# Autodesk Inventor assembly: hintererAufbau
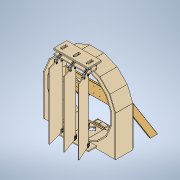
[picture p0: Inventor's stored thumbnail of the model, 180x180]
Saved by Autodesk Inventor 2020.3 (Build 243373000, 373)
## iProperties
Created: 2021-02-11
Part Number: hintererAufbau
Document SubType Name: Assembly
Designer: Stefan
Author: Stefan
## Documents named in this file (31)
- D:\Stefan\Schule\HTL\Diplomarbeit\git\Inventor\hintererAufbau\hintererAufbau.iam
- D:\Stefan\Schule\HTL\Diplomarbeit\git\Inventor\hintererAufbau\Hauptplatte.ipt
- D:\Stefan\Schule\HTL\Diplomarbeit\git\Inventor\hintererAufbau\InnenUnten.ipt
- D:\Stefan\Schule\HTL\Diplomarbeit\git\Inventor\hintererAufbau\aussenOben.ipt
- D:\Stefan\Schule\HTL\Diplomarbeit\git\Inventor\hintererAufbau\PlatteInnenEineSeite.ipt
- D:\Stefan\Schule\HTL\Diplomarbeit\git\Inventor\hintererAufbau\PlatteInnenzweiSeiten.ipt
- D:\Stefan\Schule\HTL\Diplomarbeit\git\Inventor\hintererAufbau\PlatteAussenEineSeite.ipt
- D:\Stefan\Schule\HTL\Diplomarbeit\git\Inventor\hintererAufbau\PlatteAussenZweiSeiten.ipt
- D:\Stefan\Schule\HTL\Diplomarbeit\git\Inventor\hintererAufbau\PlatteAußenGross.ipt
- D:\Stefan\Schule\HTL\Diplomarbeit\git\Inventor\3D-Druck\Fahnen_Halter_hauptteil.ipt
- D:\Stefan\Schule\HTL\Diplomarbeit\git\Inventor\3D-Druck\Fahnen_Halter_rechteck.ipt
- D:\Stefan\Schule\HTL\Diplomarbeit\git\Inventor\3D-Druck\Fahnen_Halter_obenTeileServo.ipt
- D:\Stefan\Schule\HTL\Diplomarbeit\git\Inventor\hintererAufbau\FahneHolz.ipt
- C:\Users\Stefan\Documents\Inventor\Content Center Files\R2020\de-DE\DIN EN 24 017\ISO 4017 - M5 x 30DIN EN.ipt
- C:\Users\Stefan\Documents\Inventor\Content Center Files\R2020\de-DE\ISO 4032(1)\ISO 4032 - M5DIN EN.ipt
- C:\Users\Stefan\Documents\Inventor\Content Center Files\R2020\de-DE\DIN EN 24 017\ISO 4017 - M5 x 40DIN EN.ipt
- D:\Stefan\Schule\HTL\Diplomarbeit\git\Inventor\hintererAufbau\VerstaerkungHintenMitte.ipt
- D:\Stefan\Schule\HTL\Diplomarbeit\git\Inventor\hintererAufbau\VerstaerkungHintenUnten.ipt
- D:\Stefan\Schule\HTL\Diplomarbeit\git\Inventor\hintererAufbau\VerstaerkungHintenSchraeg.ipt
- D:\Stefan\Schule\HTL\Diplomarbeit\git\Inventor\hintererAufbau\HalterungServoHochSeitlich2.ipt
- D:\Stefan\Schule\HTL\Diplomarbeit\git\Inventor\hintererAufbau\HalterungServosHochSeitlich.ipt
- D:\Stefan\Schule\HTL\Diplomarbeit\git\Inventor\hintererAufbau\HolzServoHalterHochLang.ipt
- D:\Stefan\Schule\HTL\Diplomarbeit\git\Inventor\hintererAufbau\HolzServoHalterMainPlatte1.ipt
- D:\Stefan\Schule\HTL\Diplomarbeit\git\Inventor\hintererAufbau\HolzServoHalterHinten.ipt
- D:\Stefan\Schule\HTL\Diplomarbeit\git\Inventor\Servo.ipt
- D:\Stefan\Schule\HTL\Diplomarbeit\git\Inventor\3D-Druck\Spacer_Relay v2.ipt
- D:\Stefan\Schule\HTL\Diplomarbeit\git\Inventor\hintererAufbau\VerstaerkungUnten.ipt
- D:\Stefan\Schule\HTL\Diplomarbeit\git\Inventor\hintererAufbau\KabelBoxPlatteLang.ipt
- D:\Stefan\Schule\HTL\Diplomarbeit\git\Inventor\hintererAufbau\KabelBoxPlatteKurz.ipt
- D:\Stefan\Schule\HTL\Diplomarbeit\git\Inventor\hintererAufbau\KabelBoxDeckel.ipt
- D:\Stefan\Schule\HTL\Diplomarbeit\git\Inventor\hintererAufbau\InventorOnlyInvisibleSchanierl.ipt
## Components (135 placed, 30 different names)
1. Hauptplatte:1 — Passend:1, Passend:3, Passend:5, Passend:6, Passend:9, Fluchtend:7, Passend:36, Passend:37, Fluchtend:14, Fluchtend:15, Fluchtend:16, Passend:46, Passend:47, Fluchtend:17, Passend:48, Passend:49, Passend:52, Passend:147, Fluchtend:66, Fluchtend:67
2. Hauptplatte:2 — Passend:2, Passend:4, Fluchtend:1, Passend:7, Fluchtend:2, Passend:8, Fluchtend:3, Passend:11, Passend:12, Passend:13, Passend:14, Passend:15, Passend:16, Passend:17, Passend:18, Fluchtend:4, Passend:19, Fluchtend:5, Passend:20, Passend:21, Fluchtend:6, Passend:22, Passend:23, Passend:24, Passend:25, Fluchtend:8, Passend:26, Passend:27, Fluchtend:9, Passend:28, Passend:29, Fluchtend:10, Passend:30, Passend:31, Passend:32, Fluchtend:11, Passend:33, Fluchtend:12, Passend:34, Passend:35, Fluchtend:13, Passend:38, Passend:39, Passend:40, Passend:41, Passend:42, Passend:43, Passend:44, Passend:45, Fluchtend:18, Passend:50, Passend:51, Fluchtend:19, Passend:99, Fluchtend:28, Fluchtend:29, Fluchtend:30, Passend:135, Fluchtend:52, Passend:148
3. InnenUnten:1 — Passend:1, Passend:2, Passend:3, Passend:4, Fluchtend:1, Passend:5, Passend:10, Passend:55, Passend:56, Passend:58, Passend:62, Passend:63, Passend:64, Passend:131, Passend:132, Passend:133, Passend:134
4. aussenOben:1 — Passend:6, Passend:7, Fluchtend:2, Passend:8, Passend:70, Passend:71, Passend:72, Passend:73, Passend:74, Passend:75, Passend:78, Passend:79, Passend:80, Passend:124, Fluchtend:49, Fluchtend:50
5. FahneHolz:1 — Passend:85, Passend:86, Passend:87, Passend:88
6. FahneHolz:2 — Passend:89, Passend:90, Passend:91, Passend:92
7. FahneHolz:3 — Passend:93, Passend:94, Passend:95, Passend:96
8. VerstaerkungHintenMitte:1 — Passend:97, Passend:98, Fluchtend:24, Fluchtend:25, Fluchtend:26, Fluchtend:27, Passend:99, Fluchtend:28, Passend:100, Fluchtend:31, Passend:101, Fluchtend:33
9. VerstaerkungHintenUnten:1 — Passend:98, Fluchtend:25, Fluchtend:27, Fluchtend:29, Fluchtend:34
10. VerstaerkungHintenUnten:2 — Passend:97, Fluchtend:24, Fluchtend:26, Fluchtend:30, Passend:136
11. VerstaerkungHintenSchraeg:1 — Passend:100, Fluchtend:31, Fluchtend:32
12. VerstaerkungHintenSchraeg:2 — Passend:101, Fluchtend:33, Fluchtend:34
13. HalterungServoHochSeitlich2:1 — Passend:104, Fluchtend:39, Passend:105, Passend:106, Passend:109, Fluchtend:42, Passend:111
14. HalterungServosHochSeitlich:1 — Passend:102, Fluchtend:35, Fluchtend:36, Fluchtend:50, Fluchtend:46
15. HolzServoHalterHochLang:1 — Passend:102, Fluchtend:35, Fluchtend:36, Passend:103, Fluchtend:37, Fluchtend:38, Passend:104, Fluchtend:39, Passend:105, Passend:106, Passend:107, Fluchtend:40, Passend:108, Passend:113, Fluchtend:49
16. HolzServoHalterMainPlatte1:1 — Fluchtend:47, Fluchtend:48, Passend:114, Passend:128, Passend:129, Passend:130
17. HalterungServoHochSeitlich2:2 — Passend:107, Fluchtend:40, Passend:108, Passend:110, Fluchtend:41, Fluchtend:43
18. HalterungServosHochSeitlich:2 — Passend:103, Fluchtend:37, Fluchtend:38
19. HolzServoHalterMainPlatte1:2 — Passend:112, Passend:113, Fluchtend:46, Fluchtend:47, Fluchtend:48, Passend:114, Passend:115, Passend:118, Passend:119, Fluchtend:51, Passend:125, Passend:126, Passend:127
20. HolzServoHalterHinten:1 — Passend:109, Passend:110, Fluchtend:41, Fluchtend:42, Passend:111, Fluchtend:43, Passend:112, Passend:124, Fluchtend:51
21. Servo:1 — Passend:115, Passend:125, Passend:128
22. Servo:2 — Passend:118, Passend:126, Passend:129
23. Servo:3 — Passend:119, Passend:127, Passend:130
24. Spacer_Relay v2:1 — Passend:131, Passend:134
25. Spacer_Relay v2:2 — Passend:132, Passend:133
26. VerstaerkungUnten:1 — Passend:135, Fluchtend:52, Passend:136, Passend:146, Fluchtend:63
27. KabelBoxPlatteLang:1 — Passend:138, Fluchtend:55, Fluchtend:56, Fluchtend:58, Passend:140, Passend:144
28. KabelBoxPlatteLang:2 — Passend:137, Fluchtend:53, Fluchtend:54, Passend:139, Fluchtend:57, Passend:146, Fluchtend:63
29. KabelBoxPlatteKurz:1 — Passend:139, Fluchtend:57, Fluchtend:58, Passend:142, Fluchtend:65
30. KabelBoxPlatteKurz:2 — Passend:137, Fluchtend:53, Fluchtend:54, Passend:138, Fluchtend:55, Fluchtend:56, Passend:145
31. KabelBoxDeckel:1 — Passend:140, Passend:141, Fluchtend:59, Fluchtend:60
32. InventorOnlyInvisibleSchanierl:1 — Passend:141, Fluchtend:59, Fluchtend:60, Passend:142
33. InventorOnlyInvisibleSchanierl:2 — Passend:143, Fluchtend:61, Fluchtend:62, Passend:145
34. KabelBoxDeckel:2 — Passend:143, Fluchtend:61, Fluchtend:62, Passend:144
35. PlatteInnenEineSeite:1 — Passend:9, Fluchtend:3, Passend:10
36. PlatteInnenEineSeite:2 — Passend:14, Passend:16
37. PlatteInnenEineSeite:3 — Passend:13, Passend:15
38. PlatteInnenEineSeite:4 — Passend:11, Passend:12
39. PlatteInnenEineSeite:5 — Passend:17, Passend:18, Fluchtend:4
40. PlatteInnenEineSeite:6 — Passend:21, Fluchtend:6, Passend:22
41. PlatteInnenEineSeite:7 — Passend:23, Fluchtend:7, Passend:24
42. PlatteInnenEineSeite:8 — Passend:27, Fluchtend:9, Passend:28
43. PlatteInnenEineSeite:9 — Passend:31, Passend:32, Fluchtend:11
44. PlatteInnenEineSeite:10 — Passend:35, Passend:36, Fluchtend:13
45. PlatteInnenEineSeite:19 — Passend:33, Fluchtend:12, Passend:34
46. PlatteInnenEineSeite:20 — Passend:29, Fluchtend:10, Passend:30
47. PlatteInnenEineSeite:21 — Passend:25, Fluchtend:8, Passend:26
48. PlatteInnenEineSeite:23 — Passend:19, Fluchtend:5, Passend:20
49. PlatteInnenzweiSeiten:1 — Passend:37, Fluchtend:14, Passend:38
50. PlatteAussenEineSeite:1 — Passend:39, Passend:40
51. PlatteAussenEineSeite:2 — Passend:41, Passend:42
52. PlatteAussenEineSeite:3 — Passend:45, Fluchtend:16, Passend:46
53. PlatteAussenEineSeite:4 — Passend:43, Fluchtend:15, Passend:44
54. PlatteAussenZweiSeiten:1 — Passend:47, Fluchtend:17, Passend:48
55. PlatteAussenZweiSeiten:2 — Passend:49, Fluchtend:18, Passend:50
56. PlatteAußenGross:1 — Passend:147, Passend:148, Fluchtend:66, Fluchtend:67
57. PlatteAußenGross:2 — Passend:51, Passend:52, Fluchtend:19, Fluchtend:32, Fluchtend:65
58. Fahnen_Halter_hauptteil:1 — Passend:56, Passend:58, Passend:61, Passend:65, Fluchtend:21, Passend:92, Einfügen:20, Einfügen:21, Einfügen:22, Einfügen:23, Einfügen:51, Einfügen:52, Einfügen:53, Einfügen:54
59. Fahnen_Halter_rechteck:1 — Passend:68, Passend:69, Fluchtend:23, Einfügen:58, Einfügen:61
60. Fahnen_Halter_hauptteil:2 — Passend:55, Passend:64, Passend:66, Passend:67, Fluchtend:22, Passend:86, Passend:87, Einfügen:24, Einfügen:25, Einfügen:26, Einfügen:27, Einfügen:28, Einfügen:29, Einfügen:30, Einfügen:31
61. Fahnen_Halter_rechteck:2 — Passend:66, Passend:67, Fluchtend:22, Einfügen:60, Einfügen:63
62. Fahnen_Halter_hauptteil:3 — Passend:62, Passend:63, Passend:68, Passend:69, Fluchtend:23, Passend:96, Einfügen:16, Einfügen:17, Einfügen:18, Einfügen:19, Einfügen:47, Einfügen:48, Einfügen:49, Einfügen:50
63. Fahnen_Halter_rechteck:3 — Passend:61, Passend:65, Fluchtend:21, Einfügen:59, Einfügen:62
64. Fahnen_Halter_hauptteil:4 — Passend:70, Passend:71, Passend:82, Passend:84, Passend:85, Einfügen:4, Einfügen:5, Einfügen:6, Einfügen:7, Einfügen:32, Einfügen:33, Einfügen:34, Einfügen:35
65. Fahnen_Halter_obenTeileServo:1 — Passend:76, Passend:77, Passend:78, Passend:94, Einfügen:1, Einfügen:46, Einfügen:55, Einfügen:66
66. Fahnen_Halter_hauptteil:5 — Passend:73, Passend:75, Passend:76, Passend:77, Passend:93, Passend:95, Einfügen:12, Einfügen:13, Einfügen:14, Einfügen:15, Einfügen:42, Einfügen:43, Einfügen:44, Einfügen:45
67. Fahnen_Halter_obenTeileServo:2 — Passend:80, Passend:82, Passend:84, Passend:88, Einfügen:3, Einfügen:36, Einfügen:57, Einfügen:64
68. Fahnen_Halter_hauptteil:6 — Passend:72, Passend:74, Passend:81, Passend:83, Passend:89, Passend:90, Einfügen:8, Einfügen:9, Einfügen:10, Einfügen:11, Einfügen:38, Einfügen:39, Einfügen:40, Einfügen:41
69. Fahnen_Halter_obenTeileServo:3 — Passend:79, Passend:81, Passend:83, Passend:91, Einfügen:2, Einfügen:37, Einfügen:56, Einfügen:65
70. DIN EN 24017 M5 x 30:1 — Einfügen:1
71. DIN EN 24017 M5 x 40:1 — Einfügen:55
72. DIN EN 24017 M5 x 40:2 — Einfügen:56
73. DIN EN 24017 M5 x 40:3 — Einfügen:57
74. DIN EN 24017 M5 x 40:4 — Einfügen:58
75. DIN EN 24017 M5 x 40:5 — Einfügen:59
76. DIN EN 24017 M5 x 40:6 — Einfügen:60
77. DIN EN 24017 M5 x 30:2 — Einfügen:2
78. DIN EN 24017 M5 x 30:3 — Einfügen:3
79. DIN EN 24017 M5 x 30:4 — Einfügen:4
80. DIN EN 24017 M5 x 30:5 — Einfügen:5
81. DIN EN 24017 M5 x 30:6 — Einfügen:6
82. DIN EN 24017 M5 x 30:7 — Einfügen:7
83. DIN EN 24017 M5 x 30:8 — Einfügen:8
84. DIN EN 24017 M5 x 30:9 — Einfügen:9
85. DIN EN 24017 M5 x 30:10 — Einfügen:10
86. DIN EN 24017 M5 x 30:11 — Einfügen:11
87. DIN EN 24017 M5 x 30:12 — Einfügen:12
88. DIN EN 24017 M5 x 30:13 — Einfügen:13
89. DIN EN 24017 M5 x 30:14 — Einfügen:14
90. DIN EN 24017 M5 x 30:15 — Einfügen:15
91. DIN EN 24017 M5 x 30:16 — Einfügen:16
92. DIN EN 24017 M5 x 30:17 — Einfügen:17
93. DIN EN 24017 M5 x 30:18 — Einfügen:18
94. DIN EN 24017 M5 x 30:19 — Einfügen:19
95. DIN EN 24017 M5 x 30:20 — Einfügen:20
96. DIN EN 24017 M5 x 30:21 — Einfügen:21
97. DIN EN 24017 M5 x 30:22 — Einfügen:22
98. DIN EN 24017 M5 x 30:23 — Einfügen:23
99. DIN EN 24017 M5 x 30:24 — Einfügen:24
100. DIN EN 24017 M5 x 30:25 — Einfügen:25
101. DIN EN 24017 M5 x 30:26 — Einfügen:26
102. DIN EN 24017 M5 x 30:27 — Einfügen:27
103. DIN EN 24032 M5:1 — Einfügen:28
104. DIN EN 24032 M5:2 — Einfügen:29
105. DIN EN 24032 M5:3 — Einfügen:30
106. DIN EN 24032 M5:4 — Einfügen:31
107. DIN EN 24032 M5:5 — Einfügen:32
108. DIN EN 24032 M5:6 — Einfügen:33
109. DIN EN 24032 M5:7 — Einfügen:34
110. DIN EN 24032 M5:8 — Einfügen:35
111. DIN EN 24032 M5:9 — Einfügen:36
112. DIN EN 24032 M5:10 — Einfügen:37
113. DIN EN 24032 M5:11 — Einfügen:38
114. DIN EN 24032 M5:12 — Einfügen:39
115. DIN EN 24032 M5:13 — Einfügen:40
116. DIN EN 24032 M5:14 — Einfügen:41
117. DIN EN 24032 M5:15 — Einfügen:42
118. DIN EN 24032 M5:16 — Einfügen:43
119. DIN EN 24032 M5:17 — Einfügen:44
120. DIN EN 24032 M5:18 — Einfügen:45
121. DIN EN 24032 M5:19 — Einfügen:46
122. DIN EN 24032 M5:20 — Einfügen:47
123. DIN EN 24032 M5:21 — Einfügen:48
124. DIN EN 24032 M5:22 — Einfügen:49
125. DIN EN 24032 M5:23 — Einfügen:50
126. DIN EN 24032 M5:24 — Einfügen:51
127. DIN EN 24032 M5:25 — Einfügen:52
128. DIN EN 24032 M5:26 — Einfügen:53
129. DIN EN 24032 M5:28 — Einfügen:61
130. DIN EN 24032 M5:29 — Einfügen:62
131. DIN EN 24032 M5:30 — Einfügen:63
132. DIN EN 24032 M5:31 — Einfügen:64
133. DIN EN 24032 M5:32 — Einfügen:65
134. DIN EN 24032 M5:33 — Einfügen:66
135. DIN EN 24032 M5:27 — Einfügen:54
## Relationships (266: Mate 137, Insert 66, Flush 63)
- Passend:1 [Mate]: Hauptplatte:1 ↔ InnenUnten:1
- Passend:2 [Mate]: Hauptplatte:2 ↔ InnenUnten:1
- Passend:3 [Mate]: Hauptplatte:1 ↔ InnenUnten:1
- Passend:4 [Mate]: Hauptplatte:2 ↔ InnenUnten:1
- Fluchtend:1 [Flush]: Hauptplatte:2 ↔ InnenUnten:1
- Passend:5 [Mate]: Hauptplatte:1 ↔ InnenUnten:1
- Passend:6 [Mate]: Hauptplatte:1 ↔ aussenOben:1
- Passend:7 [Mate]: Hauptplatte:2 ↔ aussenOben:1
- Fluchtend:2 [Flush]: Hauptplatte:2 ↔ aussenOben:1
- Passend:8 [Mate]: Hauptplatte:2 ↔ aussenOben:1
- Passend:9 [Mate]: Hauptplatte:1 ↔ PlatteInnenEineSeite:1
- Fluchtend:3 [Flush]: Hauptplatte:2 ↔ PlatteInnenEineSeite:1
- Passend:10 [Mate]: InnenUnten:1 ↔ PlatteInnenEineSeite:1
- Passend:11 [Mate]: Hauptplatte:2 ↔ PlatteInnenEineSeite:4
- Passend:12 [Mate]: Hauptplatte:2 ↔ PlatteInnenEineSeite:4
- Passend:13 [Mate]: Hauptplatte:2 ↔ PlatteInnenEineSeite:3
- Passend:14 [Mate]: Hauptplatte:2 ↔ PlatteInnenEineSeite:2
- Passend:15 [Mate]: Hauptplatte:2 ↔ PlatteInnenEineSeite:3
- Passend:16 [Mate]: Hauptplatte:2 ↔ PlatteInnenEineSeite:2
- Passend:17 [Mate]: Hauptplatte:2 ↔ PlatteInnenEineSeite:5
- Passend:18 [Mate]: Hauptplatte:2 ↔ PlatteInnenEineSeite:5
- Fluchtend:4 [Flush]: Hauptplatte:2 ↔ PlatteInnenEineSeite:5
- Passend:19 [Mate]: Hauptplatte:2 ↔ PlatteInnenEineSeite:23
- Fluchtend:5 [Flush]: Hauptplatte:2 ↔ PlatteInnenEineSeite:23
- Passend:20 [Mate]: Hauptplatte:2 ↔ PlatteInnenEineSeite:23
- Passend:21 [Mate]: Hauptplatte:2 ↔ PlatteInnenEineSeite:6
- Fluchtend:6 [Flush]: Hauptplatte:2 ↔ PlatteInnenEineSeite:6
- Passend:22 [Mate]: Hauptplatte:2 ↔ PlatteInnenEineSeite:6
- Passend:23 [Mate]: Hauptplatte:2 ↔ PlatteInnenEineSeite:7
- Fluchtend:7 [Flush]: Hauptplatte:1 ↔ PlatteInnenEineSeite:7
- Passend:24 [Mate]: Hauptplatte:2 ↔ PlatteInnenEineSeite:7
- Passend:25 [Mate]: Hauptplatte:2 ↔ PlatteInnenEineSeite:21
- Fluchtend:8 [Flush]: Hauptplatte:2 ↔ PlatteInnenEineSeite:21
- Passend:26 [Mate]: Hauptplatte:2 ↔ PlatteInnenEineSeite:21
- Passend:27 [Mate]: Hauptplatte:2 ↔ PlatteInnenEineSeite:8
- Fluchtend:9 [Flush]: Hauptplatte:2 ↔ PlatteInnenEineSeite:8
- Passend:28 [Mate]: Hauptplatte:2 ↔ PlatteInnenEineSeite:8
- Passend:29 [Mate]: Hauptplatte:2 ↔ PlatteInnenEineSeite:20
- Fluchtend:10 [Flush]: Hauptplatte:2 ↔ PlatteInnenEineSeite:20
- Passend:30 [Mate]: Hauptplatte:2 ↔ PlatteInnenEineSeite:20
- Passend:31 [Mate]: Hauptplatte:2 ↔ PlatteInnenEineSeite:9
- Passend:32 [Mate]: Hauptplatte:2 ↔ PlatteInnenEineSeite:9
- Fluchtend:11 [Flush]: Hauptplatte:2 ↔ PlatteInnenEineSeite:9
- Passend:33 [Mate]: Hauptplatte:2 ↔ PlatteInnenEineSeite:19
- Fluchtend:12 [Flush]: Hauptplatte:2 ↔ PlatteInnenEineSeite:19
- Passend:34 [Mate]: Hauptplatte:2 ↔ PlatteInnenEineSeite:19
- Passend:35 [Mate]: Hauptplatte:2 ↔ PlatteInnenEineSeite:10
- Passend:36 [Mate]: Hauptplatte:1 ↔ PlatteInnenEineSeite:10
- Fluchtend:13 [Flush]: Hauptplatte:2 ↔ PlatteInnenEineSeite:10
- Passend:37 [Mate]: Hauptplatte:1 ↔ PlatteInnenzweiSeiten:1
- Fluchtend:14 [Flush]: Hauptplatte:1 ↔ PlatteInnenzweiSeiten:1
- Passend:38 [Mate]: Hauptplatte:2 ↔ PlatteInnenzweiSeiten:1
- Passend:39 [Mate]: Hauptplatte:2 ↔ PlatteAussenEineSeite:1
- Passend:40 [Mate]: Hauptplatte:2 ↔ PlatteAussenEineSeite:1
- Passend:41 [Mate]: Hauptplatte:2 ↔ PlatteAussenEineSeite:2
- Passend:42 [Mate]: Hauptplatte:2 ↔ PlatteAussenEineSeite:2
- Passend:43 [Mate]: Hauptplatte:2 ↔ PlatteAussenEineSeite:4
- Fluchtend:15 [Flush]: Hauptplatte:1 ↔ PlatteAussenEineSeite:4
- Passend:44 [Mate]: Hauptplatte:2 ↔ PlatteAussenEineSeite:4
- Passend:45 [Mate]: Hauptplatte:2 ↔ PlatteAussenEineSeite:3
- Fluchtend:16 [Flush]: Hauptplatte:1 ↔ PlatteAussenEineSeite:3
- Passend:46 [Mate]: Hauptplatte:1 ↔ PlatteAussenEineSeite:3
- Passend:47 [Mate]: Hauptplatte:1 ↔ PlatteAussenZweiSeiten:1
- Fluchtend:17 [Flush]: Hauptplatte:1 ↔ PlatteAussenZweiSeiten:1
- Passend:48 [Mate]: Hauptplatte:1 ↔ PlatteAussenZweiSeiten:1
- Passend:49 [Mate]: Hauptplatte:1 ↔ PlatteAussenZweiSeiten:2
- Fluchtend:18 [Flush]: Hauptplatte:2 ↔ PlatteAussenZweiSeiten:2
- Passend:50 [Mate]: Hauptplatte:2 ↔ PlatteAussenZweiSeiten:2
- Passend:51 [Mate]: Hauptplatte:2 ↔ PlatteAußenGross:2
- Passend:52 [Mate]: Hauptplatte:1 ↔ PlatteAußenGross:2
- Fluchtend:19 [Flush]: Hauptplatte:2 ↔ PlatteAußenGross:2
- Passend:55 [Mate]: InnenUnten:1 ↔ Fahnen_Halter_hauptteil:2
- Passend:56 [Mate]: InnenUnten:1 ↔ Fahnen_Halter_hauptteil:1
- Passend:58 [Mate] (0.15 mm): InnenUnten:1 ↔ Fahnen_Halter_hauptteil:1
- Passend:61 [Mate]: Fahnen_Halter_hauptteil:1 ↔ Fahnen_Halter_rechteck:3
- Passend:62 [Mate]: InnenUnten:1 ↔ Fahnen_Halter_hauptteil:3
- Passend:63 [Mate] (0.15 mm): InnenUnten:1 ↔ Fahnen_Halter_hauptteil:3
- Passend:64 [Mate]: InnenUnten:1 ↔ Fahnen_Halter_hauptteil:2
- Passend:65 [Mate] (0.25 mm): Fahnen_Halter_hauptteil:1 ↔ Fahnen_Halter_rechteck:3
- Fluchtend:21 [Flush]: Fahnen_Halter_hauptteil:1 ↔ Fahnen_Halter_rechteck:3
- Passend:66 [Mate]: Fahnen_Halter_hauptteil:2 ↔ Fahnen_Halter_rechteck:2
- Passend:67 [Mate] (0.25 mm): Fahnen_Halter_hauptteil:2 ↔ Fahnen_Halter_rechteck:2
- Fluchtend:22 [Flush]: Fahnen_Halter_hauptteil:2 ↔ Fahnen_Halter_rechteck:2
- Passend:68 [Mate]: Fahnen_Halter_rechteck:1 ↔ Fahnen_Halter_hauptteil:3
- Passend:69 [Mate] (0.25 mm): Fahnen_Halter_rechteck:1 ↔ Fahnen_Halter_hauptteil:3
- Fluchtend:23 [Flush]: Fahnen_Halter_rechteck:1 ↔ Fahnen_Halter_hauptteil:3
- Passend:70 [Mate]: aussenOben:1 ↔ Fahnen_Halter_hauptteil:4
- Passend:71 [Mate] (0.15 mm): aussenOben:1 ↔ Fahnen_Halter_hauptteil:4
- Passend:72 [Mate]: aussenOben:1 ↔ Fahnen_Halter_hauptteil:6
- Passend:73 [Mate]: aussenOben:1 ↔ Fahnen_Halter_hauptteil:5
- Passend:74 [Mate] (0.15 mm): aussenOben:1 ↔ Fahnen_Halter_hauptteil:6
- Passend:75 [Mate] (0.15 mm): aussenOben:1 ↔ Fahnen_Halter_hauptteil:5
- Passend:76 [Mate]: Fahnen_Halter_obenTeileServo:1 ↔ Fahnen_Halter_hauptteil:5
- Passend:77 [Mate] (0.25 mm): Fahnen_Halter_obenTeileServo:1 ↔ Fahnen_Halter_hauptteil:5
- Passend:78 [Mate] (0.15 mm): aussenOben:1 ↔ Fahnen_Halter_obenTeileServo:1
- Passend:79 [Mate] (0.15 mm): aussenOben:1 ↔ Fahnen_Halter_obenTeileServo:3
- Passend:80 [Mate] (0.15 mm): aussenOben:1 ↔ Fahnen_Halter_obenTeileServo:2
- Passend:81 [Mate]: Fahnen_Halter_hauptteil:6 ↔ Fahnen_Halter_obenTeileServo:3
- Passend:82 [Mate]: Fahnen_Halter_hauptteil:4 ↔ Fahnen_Halter_obenTeileServo:2
- Passend:83 [Mate] (0.25 mm): Fahnen_Halter_hauptteil:6 ↔ Fahnen_Halter_obenTeileServo:3
- Passend:84 [Mate] (0.25 mm): Fahnen_Halter_hauptteil:4 ↔ Fahnen_Halter_obenTeileServo:2
- Passend:85 [Mate]: FahneHolz:1 ↔ Fahnen_Halter_hauptteil:4
- Passend:86 [Mate]: FahneHolz:1 ↔ Fahnen_Halter_hauptteil:2
- Passend:87 [Mate] (0.15 mm): FahneHolz:1 ↔ Fahnen_Halter_hauptteil:2
- Passend:88 [Mate]: FahneHolz:1 ↔ Fahnen_Halter_obenTeileServo:2
- Passend:89 [Mate]: FahneHolz:2 ↔ Fahnen_Halter_hauptteil:6
- Passend:90 [Mate] (0.15 mm): FahneHolz:2 ↔ Fahnen_Halter_hauptteil:6
- Passend:91 [Mate]: FahneHolz:2 ↔ Fahnen_Halter_obenTeileServo:3
- Passend:92 [Mate] (0.15 mm): FahneHolz:2 ↔ Fahnen_Halter_hauptteil:1
- Passend:93 [Mate]: FahneHolz:3 ↔ Fahnen_Halter_hauptteil:5
- Passend:94 [Mate]: FahneHolz:3 ↔ Fahnen_Halter_obenTeileServo:1
- Passend:95 [Mate] (0.15 mm): FahneHolz:3 ↔ Fahnen_Halter_hauptteil:5
- Passend:96 [Mate] (0.15 mm): FahneHolz:3 ↔ Fahnen_Halter_hauptteil:3
- Einfügen:1 [Insert]: Fahnen_Halter_obenTeileServo:1 ↔ DIN EN 24017 M5 x 30:1
- Einfügen:2 [Insert]: Fahnen_Halter_obenTeileServo:3 ↔ DIN EN 24017 M5 x 30:2
- Einfügen:3 [Insert]: Fahnen_Halter_obenTeileServo:2 ↔ DIN EN 24017 M5 x 30:3
- Einfügen:4 [Insert]: Fahnen_Halter_hauptteil:4 ↔ DIN EN 24017 M5 x 30:4
- Einfügen:5 [Insert]: Fahnen_Halter_hauptteil:4 ↔ DIN EN 24017 M5 x 30:5
- Einfügen:6 [Insert]: Fahnen_Halter_hauptteil:4 ↔ DIN EN 24017 M5 x 30:6
- Einfügen:7 [Insert]: Fahnen_Halter_hauptteil:4 ↔ DIN EN 24017 M5 x 30:7
- Einfügen:8 [Insert]: Fahnen_Halter_hauptteil:6 ↔ DIN EN 24017 M5 x 30:8
- Einfügen:9 [Insert]: Fahnen_Halter_hauptteil:6 ↔ DIN EN 24017 M5 x 30:9
- Einfügen:10 [Insert]: Fahnen_Halter_hauptteil:6 ↔ DIN EN 24017 M5 x 30:10
- Einfügen:11 [Insert]: Fahnen_Halter_hauptteil:6 ↔ DIN EN 24017 M5 x 30:11
- Einfügen:12 [Insert]: Fahnen_Halter_hauptteil:5 ↔ DIN EN 24017 M5 x 30:12
- Einfügen:13 [Insert]: Fahnen_Halter_hauptteil:5 ↔ DIN EN 24017 M5 x 30:13
- Einfügen:14 [Insert]: Fahnen_Halter_hauptteil:5 ↔ DIN EN 24017 M5 x 30:14
- Einfügen:15 [Insert]: Fahnen_Halter_hauptteil:5 ↔ DIN EN 24017 M5 x 30:15
- Einfügen:16 [Insert]: Fahnen_Halter_hauptteil:3 ↔ DIN EN 24017 M5 x 30:16
- Einfügen:17 [Insert]: Fahnen_Halter_hauptteil:3 ↔ DIN EN 24017 M5 x 30:17
- Einfügen:18 [Insert]: Fahnen_Halter_hauptteil:3 ↔ DIN EN 24017 M5 x 30:18
- Einfügen:19 [Insert]: Fahnen_Halter_hauptteil:3 ↔ DIN EN 24017 M5 x 30:19
- Einfügen:20 [Insert]: Fahnen_Halter_hauptteil:1 ↔ DIN EN 24017 M5 x 30:20
- Einfügen:21 [Insert]: Fahnen_Halter_hauptteil:1 ↔ DIN EN 24017 M5 x 30:21
- Einfügen:22 [Insert]: Fahnen_Halter_hauptteil:1 ↔ DIN EN 24017 M5 x 30:22
- Einfügen:23 [Insert]: Fahnen_Halter_hauptteil:1 ↔ DIN EN 24017 M5 x 30:23
- Einfügen:24 [Insert]: Fahnen_Halter_hauptteil:2 ↔ DIN EN 24017 M5 x 30:24
- Einfügen:25 [Insert]: Fahnen_Halter_hauptteil:2 ↔ DIN EN 24017 M5 x 30:25
- Einfügen:26 [Insert]: Fahnen_Halter_hauptteil:2 ↔ DIN EN 24017 M5 x 30:26
- Einfügen:27 [Insert]: Fahnen_Halter_hauptteil:2 ↔ DIN EN 24017 M5 x 30:27
- Einfügen:28 [Insert]: Fahnen_Halter_hauptteil:2 ↔ DIN EN 24032 M5:1
- Einfügen:29 [Insert]: Fahnen_Halter_hauptteil:2 ↔ DIN EN 24032 M5:2
- Einfügen:30 [Insert]: Fahnen_Halter_hauptteil:2 ↔ DIN EN 24032 M5:3
- Einfügen:31 [Insert]: Fahnen_Halter_hauptteil:2 ↔ DIN EN 24032 M5:4
- Einfügen:32 [Insert]: Fahnen_Halter_hauptteil:4 ↔ DIN EN 24032 M5:5
- Einfügen:33 [Insert]: Fahnen_Halter_hauptteil:4 ↔ DIN EN 24032 M5:6
- Einfügen:34 [Insert]: Fahnen_Halter_hauptteil:4 ↔ DIN EN 24032 M5:7
- Einfügen:35 [Insert]: Fahnen_Halter_hauptteil:4 ↔ DIN EN 24032 M5:8
- Einfügen:36 [Insert]: Fahnen_Halter_obenTeileServo:2 ↔ DIN EN 24032 M5:9
- Einfügen:37 [Insert]: Fahnen_Halter_obenTeileServo:3 ↔ DIN EN 24032 M5:10
- Einfügen:38 [Insert]: Fahnen_Halter_hauptteil:6 ↔ DIN EN 24032 M5:11
- Einfügen:39 [Insert]: Fahnen_Halter_hauptteil:6 ↔ DIN EN 24032 M5:12
- Einfügen:40 [Insert]: Fahnen_Halter_hauptteil:6 ↔ DIN EN 24032 M5:13
- Einfügen:41 [Insert]: Fahnen_Halter_hauptteil:6 ↔ DIN EN 24032 M5:14
- Einfügen:42 [Insert]: Fahnen_Halter_hauptteil:5 ↔ DIN EN 24032 M5:15
- Einfügen:43 [Insert]: Fahnen_Halter_hauptteil:5 ↔ DIN EN 24032 M5:16
- Einfügen:44 [Insert]: Fahnen_Halter_hauptteil:5 ↔ DIN EN 24032 M5:17
- Einfügen:45 [Insert]: Fahnen_Halter_hauptteil:5 ↔ DIN EN 24032 M5:18
- Einfügen:46 [Insert]: Fahnen_Halter_obenTeileServo:1 ↔ DIN EN 24032 M5:19
- Einfügen:47 [Insert]: Fahnen_Halter_hauptteil:3 ↔ DIN EN 24032 M5:20
- Einfügen:48 [Insert]: Fahnen_Halter_hauptteil:3 ↔ DIN EN 24032 M5:21
- Einfügen:49 [Insert]: Fahnen_Halter_hauptteil:3 ↔ DIN EN 24032 M5:22
- Einfügen:50 [Insert]: Fahnen_Halter_hauptteil:3 ↔ DIN EN 24032 M5:23
- Einfügen:51 [Insert]: Fahnen_Halter_hauptteil:1 ↔ DIN EN 24032 M5:24
- Einfügen:52 [Insert]: Fahnen_Halter_hauptteil:1 ↔ DIN EN 24032 M5:25
- Einfügen:53 [Insert]: Fahnen_Halter_hauptteil:1 ↔ DIN EN 24032 M5:26
- Einfügen:54 [Insert]: Fahnen_Halter_hauptteil:1 ↔ DIN EN 24032 M5:27
- Einfügen:55 [Insert]: Fahnen_Halter_obenTeileServo:1 ↔ DIN EN 24017 M5 x 40:1
- Einfügen:56 [Insert]: Fahnen_Halter_obenTeileServo:3 ↔ DIN EN 24017 M5 x 40:2
- Einfügen:57 [Insert]: Fahnen_Halter_obenTeileServo:2 ↔ DIN EN 24017 M5 x 40:3
- Einfügen:58 [Insert]: Fahnen_Halter_rechteck:1 ↔ DIN EN 24017 M5 x 40:4
- Einfügen:59 [Insert]: Fahnen_Halter_rechteck:3 ↔ DIN EN 24017 M5 x 40:5
- Einfügen:60 [Insert]: Fahnen_Halter_rechteck:2 ↔ DIN EN 24017 M5 x 40:6
- Einfügen:61 [Insert]: Fahnen_Halter_rechteck:1 ↔ DIN EN 24032 M5:28
- Einfügen:62 [Insert]: Fahnen_Halter_rechteck:3 ↔ DIN EN 24032 M5:29
- Einfügen:63 [Insert]: Fahnen_Halter_rechteck:2 ↔ DIN EN 24032 M5:30
- Einfügen:64 [Insert]: Fahnen_Halter_obenTeileServo:2 ↔ DIN EN 24032 M5:31
- Einfügen:65 [Insert]: Fahnen_Halter_obenTeileServo:3 ↔ DIN EN 24032 M5:32
- Einfügen:66 [Insert]: Fahnen_Halter_obenTeileServo:1 ↔ DIN EN 24032 M5:33
- Passend:97 [Mate]: VerstaerkungHintenMitte:1 ↔ VerstaerkungHintenUnten:2
- Passend:98 [Mate]: VerstaerkungHintenMitte:1 ↔ VerstaerkungHintenUnten:1
- Fluchtend:24 [Flush]: VerstaerkungHintenMitte:1 ↔ VerstaerkungHintenUnten:2
- Fluchtend:25 [Flush]: VerstaerkungHintenMitte:1 ↔ VerstaerkungHintenUnten:1
- Fluchtend:26 [Flush]: VerstaerkungHintenMitte:1 ↔ VerstaerkungHintenUnten:2
- Fluchtend:27 [Flush]: VerstaerkungHintenMitte:1 ↔ VerstaerkungHintenUnten:1
- Passend:99 [Mate]: Hauptplatte:2 ↔ VerstaerkungHintenMitte:1
- Fluchtend:28 [Flush] (5 mm): Hauptplatte:2 ↔ VerstaerkungHintenMitte:1
- Fluchtend:29 [Flush]: Hauptplatte:2 ↔ VerstaerkungHintenUnten:1
- Fluchtend:30 [Flush]: Hauptplatte:2 ↔ VerstaerkungHintenUnten:2
- Passend:100 [Mate]: VerstaerkungHintenMitte:1 ↔ VerstaerkungHintenSchraeg:1
- Fluchtend:31 [Flush]: VerstaerkungHintenMitte:1 ↔ VerstaerkungHintenSchraeg:1
- Fluchtend:32 [Flush]: VerstaerkungHintenSchraeg:1 ↔ PlatteAußenGross:2
- Passend:101 [Mate]: VerstaerkungHintenMitte:1 ↔ VerstaerkungHintenSchraeg:2
- Fluchtend:33 [Flush]: VerstaerkungHintenMitte:1 ↔ VerstaerkungHintenSchraeg:2
- Fluchtend:34 [Flush]: VerstaerkungHintenUnten:1 ↔ VerstaerkungHintenSchraeg:2
- Passend:102 [Mate]: HalterungServosHochSeitlich:1 ↔ HolzServoHalterHochLang:1
- Fluchtend:35 [Flush]: HalterungServosHochSeitlich:1 ↔ HolzServoHalterHochLang:1
- Fluchtend:36 [Flush]: HalterungServosHochSeitlich:1 ↔ HolzServoHalterHochLang:1
- Passend:103 [Mate]: HolzServoHalterHochLang:1 ↔ HalterungServosHochSeitlich:2
- Fluchtend:37 [Flush]: HolzServoHalterHochLang:1 ↔ HalterungServosHochSeitlich:2
- Fluchtend:38 [Flush]: HolzServoHalterHochLang:1 ↔ HalterungServosHochSeitlich:2
- Passend:104 [Mate]: HalterungServoHochSeitlich2:1 ↔ HolzServoHalterHochLang:1
- Fluchtend:39 [Flush]: HalterungServoHochSeitlich2:1 ↔ HolzServoHalterHochLang:1
- Passend:105 [Mate]: HalterungServoHochSeitlich2:1 ↔ HolzServoHalterHochLang:1
- Passend:106 [Mate]: HalterungServoHochSeitlich2:1 ↔ HolzServoHalterHochLang:1
- Passend:107 [Mate]: HolzServoHalterHochLang:1 ↔ HalterungServoHochSeitlich2:2
- Fluchtend:40 [Flush]: HolzServoHalterHochLang:1 ↔ HalterungServoHochSeitlich2:2
- Passend:108 [Mate]: HolzServoHalterHochLang:1 ↔ HalterungServoHochSeitlich2:2
- Passend:109 [Mate]: HalterungServoHochSeitlich2:1 ↔ HolzServoHalterHinten:1
- Passend:110 [Mate]: HalterungServoHochSeitlich2:2 ↔ HolzServoHalterHinten:1
- Fluchtend:41 [Flush]: HalterungServoHochSeitlich2:2 ↔ HolzServoHalterHinten:1
- Fluchtend:42 [Flush]: HalterungServoHochSeitlich2:1 ↔ HolzServoHalterHinten:1
- Passend:111 [Mate]: HalterungServoHochSeitlich2:1 ↔ HolzServoHalterHinten:1
- Fluchtend:43 [Flush]: HalterungServoHochSeitlich2:2 ↔ HolzServoHalterHinten:1
- Passend:112 [Mate]: HolzServoHalterMainPlatte1:2 ↔ HolzServoHalterHinten:1
- Passend:113 [Mate]: HolzServoHalterHochLang:1 ↔ HolzServoHalterMainPlatte1:2
- Fluchtend:46 [Flush]: HalterungServosHochSeitlich:1 ↔ HolzServoHalterMainPlatte1:2
- Fluchtend:47 [Flush]: HolzServoHalterMainPlatte1:1 ↔ HolzServoHalterMainPlatte1:2
- Fluchtend:48 [Flush]: HolzServoHalterMainPlatte1:1 ↔ HolzServoHalterMainPlatte1:2
- Passend:114 [Mate]: HolzServoHalterMainPlatte1:1 ↔ HolzServoHalterMainPlatte1:2
- Passend:115 [Mate]: HolzServoHalterMainPlatte1:2 ↔ Servo:1
- Passend:118 [Mate]: HolzServoHalterMainPlatte1:2 ↔ Servo:2
- Passend:119 [Mate]: HolzServoHalterMainPlatte1:2 ↔ Servo:3
- Passend:124 [Mate]: aussenOben:1 ↔ HolzServoHalterHinten:1
- Fluchtend:49 [Flush]: aussenOben:1 ↔ HolzServoHalterHochLang:1
- Fluchtend:50 [Flush]: aussenOben:1 ↔ HalterungServosHochSeitlich:1
- Fluchtend:51 [Flush]: HolzServoHalterMainPlatte1:2 ↔ HolzServoHalterHinten:1
- Passend:125 [Mate]: HolzServoHalterMainPlatte1:2 ↔ Servo:1
- Passend:126 [Mate]: HolzServoHalterMainPlatte1:2 ↔ Servo:2
- Passend:127 [Mate]: HolzServoHalterMainPlatte1:2 ↔ Servo:3
- Passend:128 [Mate]: HolzServoHalterMainPlatte1:1 ↔ Servo:1
- Passend:129 [Mate]: HolzServoHalterMainPlatte1:1 ↔ Servo:2
- Passend:130 [Mate]: HolzServoHalterMainPlatte1:1 ↔ Servo:3
- Passend:131 [Mate]: InnenUnten:1 ↔ Spacer_Relay v2:1
- Passend:132 [Mate]: InnenUnten:1 ↔ Spacer_Relay v2:2
- Passend:133 [Mate]: InnenUnten:1 ↔ Spacer_Relay v2:2
- Passend:134 [Mate]: InnenUnten:1 ↔ Spacer_Relay v2:1
- Passend:135 [Mate]: Hauptplatte:2 ↔ VerstaerkungUnten:1
- Fluchtend:52 [Flush]: Hauptplatte:2 ↔ VerstaerkungUnten:1
- Passend:136 [Mate]: VerstaerkungHintenUnten:2 ↔ VerstaerkungUnten:1
- Passend:137 [Mate]: KabelBoxPlatteLang:2 ↔ KabelBoxPlatteKurz:2
- Fluchtend:53 [Flush]: KabelBoxPlatteLang:2 ↔ KabelBoxPlatteKurz:2
- Fluchtend:54 [Flush]: KabelBoxPlatteLang:2 ↔ KabelBoxPlatteKurz:2
- Passend:138 [Mate]: KabelBoxPlatteLang:1 ↔ KabelBoxPlatteKurz:2
- Fluchtend:55 [Flush]: KabelBoxPlatteLang:1 ↔ KabelBoxPlatteKurz:2
- Fluchtend:56 [Flush]: KabelBoxPlatteLang:1 ↔ KabelBoxPlatteKurz:2
- Passend:139 [Mate]: KabelBoxPlatteLang:2 ↔ KabelBoxPlatteKurz:1
- Fluchtend:57 [Flush]: KabelBoxPlatteLang:2 ↔ KabelBoxPlatteKurz:1
- Fluchtend:58 [Flush]: KabelBoxPlatteLang:1 ↔ KabelBoxPlatteKurz:1
- Passend:140 [Mate]: KabelBoxPlatteLang:1 ↔ KabelBoxDeckel:1
- Passend:141 [Mate]: KabelBoxDeckel:1 ↔ InventorOnlyInvisibleSchanierl:1
- Fluchtend:59 [Flush]: KabelBoxDeckel:1 ↔ InventorOnlyInvisibleSchanierl:1
- Fluchtend:60 [Flush]: KabelBoxDeckel:1 ↔ InventorOnlyInvisibleSchanierl:1
- Passend:142 [Mate]: KabelBoxPlatteKurz:1 ↔ InventorOnlyInvisibleSchanierl:1
- Passend:143 [Mate]: InventorOnlyInvisibleSchanierl:2 ↔ KabelBoxDeckel:2
- Fluchtend:61 [Flush]: InventorOnlyInvisibleSchanierl:2 ↔ KabelBoxDeckel:2
- Fluchtend:62 [Flush]: InventorOnlyInvisibleSchanierl:2 ↔ KabelBoxDeckel:2
- Passend:144 [Mate]: KabelBoxPlatteLang:1 ↔ KabelBoxDeckel:2
- Passend:145 [Mate]: KabelBoxPlatteKurz:2 ↔ InventorOnlyInvisibleSchanierl:2
- Passend:146 [Mate]: VerstaerkungUnten:1 ↔ KabelBoxPlatteLang:2
- Fluchtend:63 [Flush]: VerstaerkungUnten:1 ↔ KabelBoxPlatteLang:2
- Fluchtend:65 [Flush] (350 mm): KabelBoxPlatteKurz:1 ↔ PlatteAußenGross:2
- Passend:147 [Mate]: Hauptplatte:1 ↔ PlatteAußenGross:1
- Passend:148 [Mate]: Hauptplatte:2 ↔ PlatteAußenGross:1
- Fluchtend:66 [Flush]: Hauptplatte:1 ↔ PlatteAußenGross:1
- Fluchtend:67 [Flush]: Hauptplatte:1 ↔ PlatteAußenGross:1
